# Autodesk Inventor assembly: Modelo
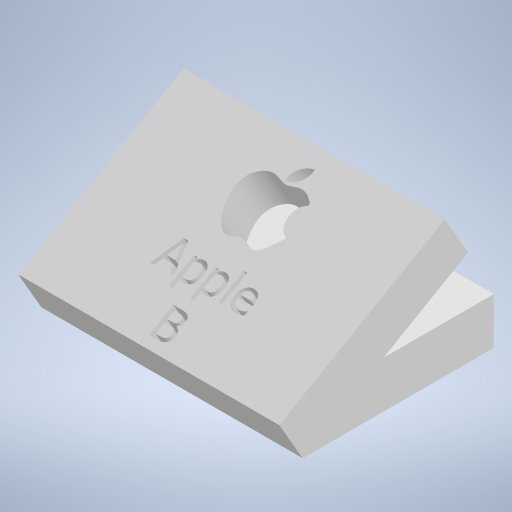
[picture p0: Inventor's stored thumbnail of the model, 512x512]
Saved by Autodesk Inventor 2023 (Build 270158000, 158)
## iProperties
Created: 2024-03-02
Part Number: Modelo
Document SubType Name: Assembly
Designer: LENOVO
Author: LENOVO
## Documents named in this file (3)
- C:\Users\LENOVO\Desktop\UN\Décimo semestre\Robótica\Laboratorios\Laboratorio 1\Modelo.iam
- C:\Users\LENOVO\Desktop\UN\Décimo semestre\Robótica\Laboratorios\Laboratorio 1\Base.ipt
- C:\Users\LENOVO\Desktop\UN\Décimo semestre\Robótica\Laboratorios\Laboratorio 1\Logo.ipt
## Components (2 placed, 2 different names)
1. Base:1 — Mate:1, Flush:1, Mate:2
2. Logo:1 — Mate:1, Flush:1, Mate:2
## Relationships (3: Mate 2, Flush 1)
- Mate:1: Base:1 ↔ Logo:1
- Flush:1: Base:1 ↔ Logo:1
- Mate:2: Base:1 ↔ Logo:1
